# Autodesk Inventor assembly: Assembly_Matchboxscope_injectionmolded
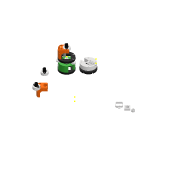
[picture p0: Inventor's stored thumbnail of the model, 180x180]
Saved by Autodesk Inventor 2022 (Build 260153000, 153)
## iProperties
Created: 2023-04-12
Part Number: Assembly_Matchboxscope_injectionmolded
Document SubType Name: Assembly
Designer: diederichbenedict
Author: diederichbenedict
## Documents named in this file (20)
- C:\Users\diederichbenedict\Dropbox\Dokumente\Promotion\PROJECTS\Matchboxscope\INVENTOR\RELEASE\InjectionMolded\Assembly_Matchboxscope_injectionmolded.iam
- C:\Users\diederichbenedict\Dropbox\Dokumente\Promotion\PROJECTS\Matchboxscope\INVENTOR\RELEASE\InjectionMolded\IM_Matchboxscope_plate.ipt
- C:\Users\diederichbenedict\Dropbox\Dokumente\Promotion\PROJECTS\Matchboxscope\INVENTOR\RELEASE\InjectionMolded\IM_Lensholder.ipt
- C:\Users\diederichbenedict\Dropbox\Dokumente\Promotion\PROJECTS\Matchboxscope\INVENTOR\RELEASE\InjectionMolded\IM_Periscope.ipt
- C:\Users\diederichbenedict\Dropbox\Dokumente\Promotion\PROJECTS\Matchboxscope\INVENTOR\RELEASE\InjectionMolded\IM_ledholder.ipt
- C:\Users\diederichbenedict\Dropbox\Dokumente\Promotion\PROJECTS\Matchboxscope\INVENTOR\RELEASE\InjectionMolded\Anglerfish_Cameraspacer.ipt
- C:\Users\diederichbenedict\Dropbox\Dokumente\Promotion\PROJECTS\Matchboxscope\INVENTOR\RELEASE\InjectionMolded\00_CCTV_M12_VCM_large.ipt
- C:\Users\diederichbenedict\Dropbox\Dokumente\Promotion\PROJECTS\Matchboxscope\INVENTOR\RELEASE\InjectionMolded\IM_Lensholder_M12.ipt
- C:\Users\diederichbenedict\Dropbox\Dokumente\Promotion\PROJECTS\Matchboxscope\INVENTOR\RELEASE\InjectionMolded\Matchboxscope_M12_Lensadapter_v0.ipt
- C:\Users\diederichbenedict\Dropbox\Dokumente\Promotion\PROJECTS\Matchboxscope\INVENTOR\RELEASE\InjectionMolded\00_Turningscrew.ipt
- C:\Users\diederichbenedict\Documents\Inventor\Content Center Files\R2022\de-DE\DIN 912\DIN 912 - M3 x 0.5 x 25 x 18.ipt
- C:\Users\diederichbenedict\Documents\Inventor\Content Center Files\R2022\de-DE\DIN 912\DIN 912 - M3 x 0.5 x 10 x 8.75.ipt
- C:\Users\diederichbenedict\Dropbox\Dokumente\Promotion\PROJECTS\Matchboxscope\INVENTOR\RELEASE\InjectionMolded\00_LED_lamp.ipt
- C:\Users\diederichbenedict\Dropbox\Dokumente\Promotion\PROJECTS\Matchboxscope\INVENTOR\RELEASE\InjectionMolded\00_Neopixel_4x4_Matrix.ipt
- C:\Users\diederichbenedict\Dropbox\Dokumente\Promotion\PROJECTS\Matchboxscope\INVENTOR\RELEASE\InjectionMolded\IM_ledmatrix_holder.ipt
- C:\Users\diederichbenedict\Dropbox\Dokumente\Promotion\PROJECTS\Matchboxscope\INVENTOR\RELEASE\InjectionMolded\IM_ledmatrix_diffuser.ipt
- C:\Users\diederichbenedict\Dropbox\Dokumente\Promotion\PROJECTS\Matchboxscope\INVENTOR\RELEASE\InjectionMolded\IM_Matchboxscope_base_old.ipt
- C:\Users\diederichbenedict\Dropbox\Dokumente\Promotion\PROJECTS\Matchboxscope\INVENTOR\RELEASE\InjectionMolded\00_toslink_launcher_v3.ipt
- C:\Users\diederichbenedict\Dropbox\Dokumente\Promotion\PROJECTS\Matchboxscope\INVENTOR\RELEASE\InjectionMolded\IM_Matchboxscope_base_xiao.ipt
- C:\Users\diederichbenedict\Dropbox\Dokumente\Promotion\PROJECTS\Matchboxscope\INVENTOR\RELEASE\InjectionMolded\IM_Matchboxscope_base_xiao_lid.ipt
## Components (32 placed, 19 different names)
1. IM_Matchboxscope_base_old:1 — Fluchtend:1, Einfügen:16, Einfügen:17, Einfügen:20, Einfügen:21, Einfügen:22, Passend:3
2. IM_Lensholder:1 — Fluchtend:1, Einfügen:8
3. IM_Periscope:1
4. IM_ledholder:1 — Einfügen:23, Einfügen:24, Winkel:3
5. Anglerfish_Cameraspacer:1
6. 00_CCTV_M12_VCM_large:1 — Passend:2, Winkel:2
7. IM_Lensholder_M12:1 — Passend:2, Winkel:2
8. Matchboxscope_M12_Lensadapter_v0:1
9. 00_Turningscrew:1 — Einfügen:21
10. DIN 912 - ersetzt durch DIN EN ISO 4762 M3 x 25:1 — Einfügen:18
11. DIN 912 - ersetzt durch DIN EN ISO 4762 M3 x 25:2
12. DIN 912 - ersetzt durch DIN EN ISO 4762 M3 x 25:3 — Einfügen:19
13. DIN 912 - ersetzt durch DIN EN ISO 4762 M3 x 10:1
14. DIN 912 - ersetzt durch DIN EN ISO 4762 M3 x 10:2
15. DIN 912 - ersetzt durch DIN EN ISO 4762 M3 x 10:3 — Einfügen:8
16. 00_Turningscrew:2 — Einfügen:20
17. 00_Turningscrew:3 — Einfügen:22
18. 00_LED_lamp:1
19. IM_Matchboxscope_plate:2 — Einfügen:17, Einfügen:18, Einfügen:19, Einfügen:23
20. 00_Neopixel_4x4_Matrix:1
21. IM_ledmatrix_holder:1 — Fluchtend:5, Fluchtend:6
22. IM_ledmatrix_diffuser:1 — Fluchtend:5, Fluchtend:6
23. IM_Matchboxscope_plate:3 — Einfügen:16
24. 00_toslink_launcher_v3:1 — Einfügen:24, Winkel:3
25. IM_ledholder:2
26. 00_toslink_launcher_v3:2
27. 00_toslink_launcher_v3:3 — Passend:3
28. 00_toslink_launcher_v3:4
29. IM_Matchboxscope_base_xiao:1 — Einfügen:25, Winkel:4, Einfügen:26, Winkel:5, Einfügen:27
30. IM_Matchboxscope_base_xiao_lid:1 — Einfügen:26, Winkel:5
31. IM_Matchboxscope_base_old:2 — Einfügen:25, Winkel:4
32. IM_Matchboxscope_plate:4 — Einfügen:27
## Relationships (22: Insert 13, Angle 4, Flush 3, Mate 2)
- Fluchtend:1 [Flush]: IM_Matchboxscope_base_old:1 ↔ IM_Lensholder:1
- Passend:2 [Mate]: 00_CCTV_M12_VCM_large:1 ↔ IM_Lensholder_M12:1
- Winkel:2 [Angle] (45 deg): 00_CCTV_M12_VCM_large:1 ↔ IM_Lensholder_M12:1
- Einfügen:8 [Insert]: IM_Lensholder:1 ↔ DIN 912 - ersetzt durch DIN EN ISO 4762 M3 x 10:3
- Fluchtend:5 [Flush]: IM_ledmatrix_holder:1 ↔ IM_ledmatrix_diffuser:1
- Fluchtend:6 [Flush]: IM_ledmatrix_holder:1 ↔ IM_ledmatrix_diffuser:1
- Einfügen:16 [Insert]: IM_Matchboxscope_base_old:1 ↔ IM_Matchboxscope_plate:3
- Einfügen:17 [Insert] (10 mm): IM_Matchboxscope_base_old:1 ↔ IM_Matchboxscope_plate:2
- Einfügen:18 [Insert]: DIN 912 - ersetzt durch DIN EN ISO 4762 M3 x 25:1 ↔ IM_Matchboxscope_plate:2
- Einfügen:19 [Insert]: DIN 912 - ersetzt durch DIN EN ISO 4762 M3 x 25:3 ↔ IM_Matchboxscope_plate:2
- Einfügen:20 [Insert]: IM_Matchboxscope_base_old:1 ↔ 00_Turningscrew:2
- Einfügen:21 [Insert]: IM_Matchboxscope_base_old:1 ↔ 00_Turningscrew:1
- Einfügen:22 [Insert]: IM_Matchboxscope_base_old:1 ↔ 00_Turningscrew:3
- Einfügen:23 [Insert]: IM_ledholder:1 ↔ IM_Matchboxscope_plate:2
- Einfügen:24 [Insert] (2 mm): IM_ledholder:1 ↔ 00_toslink_launcher_v3:1
- Winkel:3 [Angle] (0 deg): IM_ledholder:1 ↔ 00_toslink_launcher_v3:1
- Passend:3 [Mate]: IM_Matchboxscope_base_old:1 ↔ 00_toslink_launcher_v3:3
- Einfügen:25 [Insert]: IM_Matchboxscope_base_xiao:1 ↔ IM_Matchboxscope_base_old:2
- Winkel:4 [Angle] (180 deg): IM_Matchboxscope_base_xiao:1 ↔ IM_Matchboxscope_base_old:2
- Einfügen:26 [Insert]: IM_Matchboxscope_base_xiao:1 ↔ IM_Matchboxscope_base_xiao_lid:1
- Winkel:5 [Angle] (0 deg): IM_Matchboxscope_base_xiao:1 ↔ IM_Matchboxscope_base_xiao_lid:1
- Einfügen:27 [Insert] (5 mm): IM_Matchboxscope_base_xiao:1 ↔ IM_Matchboxscope_plate:4
